# Autodesk Inventor assembly: Zespół1
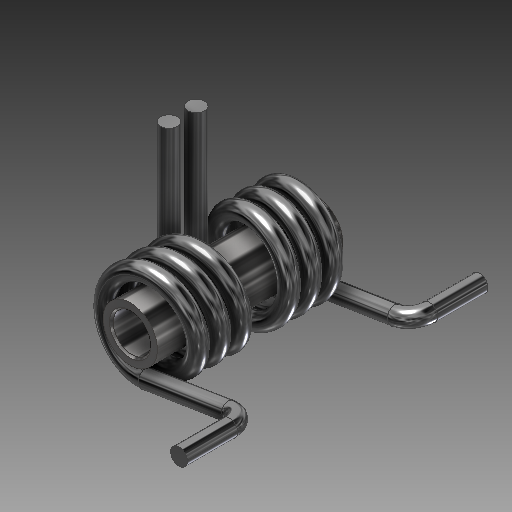
[picture p0: Inventor's stored thumbnail of the model, 512x512]
Saved by Autodesk Inventor 2017 SP1 (Build 210196100, 196)
## iProperties
Created: 2021-02-07
Part Number: Zespół1
Document SubType Name: Assembly
Designer: Napoleon
Author: Napoleon
## Documents named in this file (4)
- D:\PRYWATNE\PROJEKTY\POKÓJ\URZĄDZENIA PERYFERYJNE\DELL 1909Wf\Zespół1.iam
- D:\PRYWATNE\PROJEKTY\POKÓJ\URZĄDZENIA PERYFERYJNE\DELL 1909Wf\SPRĘŻYNA 1.ipt
- D:\PRYWATNE\PROJEKTY\POKÓJ\URZĄDZENIA PERYFERYJNE\DELL 1909Wf\SPRĘŻYNA 2.ipt
- D:\PRYWATNE\PROJEKTY\POKÓJ\URZĄDZENIA PERYFERYJNE\DELL 1909Wf\TULEJKA.ipt
## Components (3 placed, 3 different names)
1. TULEJKA:1 — Sztywne:2
2. SPRĘŻYNA 1:1 — Równoległy:1, Sztywne:1, Sztywne:2
3. SPRĘŻYNA 2:1 — Równoległy:1, Sztywne:1
## Relationships (3: WeldJoint 2, Flush 1)
- Równoległy:1 [Flush]: SPRĘŻYNA 1:1 ↔ SPRĘŻYNA 2:1
- Sztywne:1 [WeldJoint] (-41 mm): SPRĘŻYNA 1:1 ↔ SPRĘŻYNA 2:1
- Sztywne:2 [WeldJoint] (-33 mm): TULEJKA:1 ↔ SPRĘŻYNA 1:1
